# Autodesk Inventor assembly: J001819
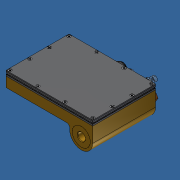
[picture p0: Inventor's stored thumbnail of the model, 180x180]
Saved by Autodesk Inventor 2012 SP2 (Build 160219200, 219)
## iProperties
Created: 2013-05-16
Vendor: HHMI: JFRC - ID&F
Document SubType Name: Assembly
Designer: JORDANJ
Project: P-48101
Description: NON-CONDENSING AIR CHILLED COOLING PLATE WITH SINTERED METAL SURFACE AND CONDENSATION DRAUGH
Part Number: J001819
RuleStatus: InUse
AfterDocSave0: file://Part Number Cleaner
DESIGN DEPARTMENT: HHMI: JFRC - ID&F
LAB/DEPT: FLY FACILITY (SHARED RESOURCE)
REQUESTING SCIENTIST: LAVERTY, TODD
SPECIAL FINISH: N/A
SURFACE ROUGHNESS: N/A
ALTERED ITEM PART NUMBER: N/A
ALTERED ITEM VENDOR: N/A
ALTERED ITEM DESCRIPTION: N/A
Revision Number: 0
## Documents named in this file (9)
- C:\_WORKSPACE\DATA\PROJECTS\COOLING APPARATUSES\NON-CONDENSING COOLING PLATE\MCAD\SIMPLE CHILLED AIR\SIMPLE CHILLED AIR NON-CONDENSING COOLING PLATE.iam
- C:\_WORKSPACE\DATA\PROJECTS\COOLING APPARATUSES\NON-CONDENSING COOLING PLATE\MCAD\SIMPLE CHILLED AIR\SIMPLE CHILLED AIR SINTERED PLATE.ipt
- C:\_WORKSPACE\DATA\PROJECTS\COOLING APPARATUSES\NON-CONDENSING COOLING PLATE\MCAD\SIMPLE CHILLED AIR\SIMPLE CHILLED AIR DRAIN PLATE.ipt
- C:\_WORKSPACE\DATA\PROJECTS\COOLING APPARATUSES\NON-CONDENSING COOLING PLATE\MCAD\SIMPLE CHILLED AIR\SIMPLE CHILLED AIR BASE PLATE.ipt
- C:\_WORKSPACE\DATA\PROJECTS\COOLING APPARATUSES\NON-CONDENSING COOLING PLATE\MCAD\COMMON\91099A167.ipt
- C:\_WORKSPACE\DATA\PROJECTS\COOLING APPARATUSES\NON-CONDENSING COOLING PLATE\MCAD\SIMPLE CHILLED AIR\SIMPLE CHILLED AIR 12mm X 17mm VIAL ADAPTER.ipt
- C:\_WORKSPACE\DATA\PROJECTS\COOLING APPARATUSES\NON-CONDENSING COOLING PLATE\MCAD\COMMON\SMC AS2211F-UO1-07.ipt
- C:\_WORKSPACE\DATA\PROJECTS\COOLING APPARATUSES\NON-CONDENSING COOLING PLATE\MCAD\SIMPLE CHILLED AIR\SIMPLE CHILLED AIR WALL FITTING.ipt
- C:\_WORKSPACE\DATA\PROJECTS\COOLING APPARATUSES\NON-CONDENSING COOLING PLATE\MCAD\COMMON\BREATHER VENT.ipt
## Components (19 placed, 8 different names)
1. SIMPLE CHILLED AIR BASE PLATE:1 — Flush:7, Flush:8, Flush:9, Insert:53, Insert:54
2. SIMPLE CHILLED AIR DRAIN PLATE:1 — Flush:4, Flush:5, Flush:6
3. SIMPLE CHILLED AIR SINTERED PLATE:1 — Flush:1, Flush:2, Flush:3, Insert:21, Insert:22, Insert:23, Insert:24, Insert:25, Insert:26, Insert:27, Insert:28, Insert:29, Insert:30, Insert:31, Insert:32
4. 91099A167:1 — Insert:21
5. 91099A167:2 — Insert:22
6. 91099A167:3 — Insert:23
7. 91099A167:4 — Insert:24
8. 91099A167:5 — Insert:25
9. 91099A167:6 — Insert:26
10. 91099A167:7 — Insert:27
11. 91099A167:8 — Insert:28
12. 91099A167:9 — Insert:29
13. 91099A167:10 — Insert:30
14. 91099A167:11 — Insert:31
15. 91099A167:12 — Insert:32
16. SIMPLE CHILLED AIR 12mm X 17mm VIAL ADAPTER:1 — Flush:13, Flush:14, Flush:15
17. SMC AS2211F-UO1-07:1 — Insert:53
18. SIMPLE CHILLED AIR WALL FITTING:1
19. BREATHER VENT:1 — Insert:54
## Relationships (26: Insert 14, Flush 12)
- Flush:1: SIMPLE CHILLED AIR SINTERED PLATE:1
- Flush:2: SIMPLE CHILLED AIR SINTERED PLATE:1
- Flush:3: SIMPLE CHILLED AIR SINTERED PLATE:1
- Flush:4: SIMPLE CHILLED AIR DRAIN PLATE:1
- Flush:5: SIMPLE CHILLED AIR DRAIN PLATE:1
- Flush:6: SIMPLE CHILLED AIR DRAIN PLATE:1
- Flush:7: SIMPLE CHILLED AIR BASE PLATE:1
- Flush:8: SIMPLE CHILLED AIR BASE PLATE:1
- Flush:9: SIMPLE CHILLED AIR BASE PLATE:1
- Flush:13: SIMPLE CHILLED AIR 12mm X 17mm VIAL ADAPTER:1
- Flush:14: SIMPLE CHILLED AIR 12mm X 17mm VIAL ADAPTER:1
- Flush:15: SIMPLE CHILLED AIR 12mm X 17mm VIAL ADAPTER:1
- Insert:53: SIMPLE CHILLED AIR BASE PLATE:1 ↔ SMC AS2211F-UO1-07:1
- Insert:54: SIMPLE CHILLED AIR BASE PLATE:1 ↔ BREATHER VENT:1
- Insert:21: SIMPLE CHILLED AIR SINTERED PLATE:1 ↔ 91099A167:1
- Insert:22: SIMPLE CHILLED AIR SINTERED PLATE:1 ↔ 91099A167:2
- Insert:23: SIMPLE CHILLED AIR SINTERED PLATE:1 ↔ 91099A167:3
- Insert:24: SIMPLE CHILLED AIR SINTERED PLATE:1 ↔ 91099A167:4
- Insert:25: SIMPLE CHILLED AIR SINTERED PLATE:1 ↔ 91099A167:5
- Insert:26: SIMPLE CHILLED AIR SINTERED PLATE:1 ↔ 91099A167:6
- Insert:27: SIMPLE CHILLED AIR SINTERED PLATE:1 ↔ 91099A167:7
- Insert:28: SIMPLE CHILLED AIR SINTERED PLATE:1 ↔ 91099A167:8
- Insert:29: SIMPLE CHILLED AIR SINTERED PLATE:1 ↔ 91099A167:9
- Insert:30: SIMPLE CHILLED AIR SINTERED PLATE:1 ↔ 91099A167:10
- Insert:31: SIMPLE CHILLED AIR SINTERED PLATE:1 ↔ 91099A167:11
- Insert:32: SIMPLE CHILLED AIR SINTERED PLATE:1 ↔ 91099A167:12
